# Autodesk Inventor assembly: cnc_3mm_v1
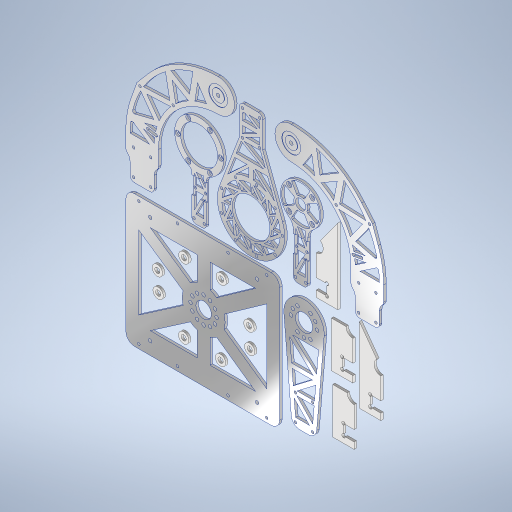
[picture p0: Inventor's stored thumbnail of the model, 512x512]
Saved by Autodesk Inventor 2024 (Build 280153000, 153)
## iProperties
Created: 2025-02-17
Part Number: cnc_3mm_v1
Document SubType Name: Assembly
Designer: tanoue_kota
Author: tanoue_kota
## Documents named in this file (12)
- C:\Users\田之上巧太\Documents\Inventor\RobArm\CNC\cnc_3mm_v1.iam
- C:\Users\田之上巧太\Documents\Inventor\RobArm\rob_link1\link1plate3.ipt
- C:\Users\田之上巧太\Documents\Inventor\RobArm\rob_link1\link1plate4.ipt
- C:\Users\田之上巧太\Documents\Inventor\RobArm\rob_link1\link1plate5.ipt
- C:\Users\田之上巧太\Documents\Inventor\RobArm\rob_link1\link1plate5_MIR.ipt
- C:\Users\田之上巧太\Documents\Inventor\RobArm\rob_link2\link2plate4.ipt
- C:\Users\田之上巧太\Documents\Inventor\RobArm\rob_link2\link2plate3.ipt
- C:\Users\田之上巧太\Documents\Inventor\RobArm\OtherParts\bendpart_36deg.ipt
- C:\Users\田之上巧太\Documents\Inventor\RobArm\OtherParts\bendpart_90deg.ipt
- C:\Users\田之上巧太\Documents\Inventor\RobArm\rob_link2\link2part8.ipt
- C:\Users\田之上巧太\Documents\Inventor\RobArm\rob_base\base_plate5.ipt
- C:\Users\田之上巧太\Documents\Inventor\RobArm\rob_base\base_part6.ipt
## Components (20 placed, 11 different names)
1. link1plate5:1
2. link1plate5_MIR:1
3. bendpart_36deg:1 — フラッシュ:4
4. bendpart_36deg:2 — フラッシュ:4
5. bendpart_90deg:1
6. bendpart_90deg:2
7. link2part8:6
8. base_plate5:1 — フラッシュ:5, フラッシュ:6, フラッシュ:7, フラッシュ:8, フラッシュ:9, フラッシュ:10, フラッシュ:11, フラッシュ:12
9. link1plate3:1
10. link1plate4:1
11. link2plate3:1
12. link2plate4:1
13. base_part6:1 — フラッシュ:8
14. base_part6:2 — フラッシュ:7
15. base_part6:3 — フラッシュ:9
16. base_part6:4 — フラッシュ:11
17. base_part6:5 — フラッシュ:12
18. base_part6:6 — フラッシュ:10
19. base_part6:7 — フラッシュ:5
20. base_part6:8 — フラッシュ:6
## Relationships (9: Flush 9)
- フラッシュ:4 [Flush]: bendpart_36deg:1 ↔ bendpart_36deg:2
- フラッシュ:5 [Flush]: base_plate5:1 ↔ base_part6:7
- フラッシュ:6 [Flush]: base_plate5:1 ↔ base_part6:8
- フラッシュ:7 [Flush]: base_plate5:1 ↔ base_part6:2
- フラッシュ:8 [Flush]: base_plate5:1 ↔ base_part6:1
- フラッシュ:9 [Flush]: base_plate5:1 ↔ base_part6:3
- フラッシュ:10 [Flush]: base_plate5:1 ↔ base_part6:6
- フラッシュ:11 [Flush]: base_plate5:1 ↔ base_part6:4
- フラッシュ:12 [Flush]: base_plate5:1 ↔ base_part6:5
